# Autodesk Inventor assembly: 2016_IEEE_SouteastCon_Court final
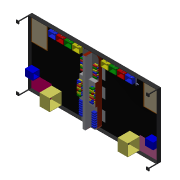
[picture p0: Inventor's stored thumbnail of the model, 180x180]
Saved by Autodesk Inventor 2015 (Build 190159000, 159)
## iProperties
Created: 2015-03-03
Part Number: 2016_IEEE_SouteastCon_Court final
Document SubType Name: Assembly
Designer: Vukica
Author: Vukica
## Documents named in this file (17)
- C:\Users\Vukica\Dropbox\IEEE\hardware rules\2016Hardware_Court_v6\2016_IEEE_SouteastCon_Court final.iam
- C:\Users\Vukica\Dropbox\IEEE\hardware rules\2016Hardware_Court_v6\Base.ipt
- C:\Users\Vukica\Dropbox\IEEE\hardware rules\2016Hardware_Court_v6\Ship area.ipt
- C:\Users\Vukica\Dropbox\IEEE\hardware rules\2016Hardware_Court_v6\Starting position pink.ipt
- C:\Users\Vukica\Dropbox\IEEE\hardware rules\2016Hardware_Court_v6\Starting position purple.ipt
- C:\Users\Vukica\Dropbox\IEEE\hardware rules\2016Hardware_Court_v6\Beacon.ipt
- C:\Users\Vukica\Dropbox\IEEE\hardware rules\2016Hardware_Court_v6\Side 84 in by 6 in by half inch.ipt
- C:\Users\Vukica\Dropbox\IEEE\hardware rules\2016Hardware_Court_v6\Side 120 in by 6 in by half inch.ipt
- C:\Users\Vukica\Dropbox\IEEE\hardware rules\2016Hardware_Court_v6\Hill.ipt
- C:\Users\Vukica\Dropbox\IEEE\hardware rules\2016Hardware_Court_v6\Blue truck.ipt
- C:\Users\Vukica\Dropbox\IEEE\hardware rules\2016Hardware_Court_v6\Tunnel.ipt
- C:\Users\Vukica\Dropbox\IEEE\hardware rules\2016Hardware_Court_v6\Shipping goods QR subassembly.iam
- C:\Users\Vukica\Dropbox\IEEE\hardware rules\2016Hardware_Court_v6\Shipping goods generic subassembly.iam
- C:\Users\Vukica\Dropbox\IEEE\hardware rules\2016Hardware_Court_v6\Shipping goods colors subassembly.iam
- C:\Users\Vukica\Dropbox\IEEE\hardware rules\2016Hardware_Court_v6\Rail truck area subassembly v2.iam
- C:\Users\Vukica\Dropbox\IEEE\hardware rules\2016Hardware_Court_v6\LED Bacon.iam
- C:\Users\Vukica\Dropbox\IEEE\hardware rules\2016Hardware_Court_v6\Stripes on the floor.ipt
## Components (31 placed, 16 different names)
1. Base:1 — Mate:1, Mate:2, Mate:3, Flush:5, Flush:6, Mate:4, Flush:7, Flush:8, Flush:11, Mate:9, Flush:12, Flush:13, Flush:15, Mate:10, Mate:11, Flush:16, Flush:18, Mate:12, Mate:17, Mate:22, Mate:30, Mate:62, Mate:125, Mate:126, Mate:127, Mate:136, Mate:137, Flush:55, Flush:56
2. Ship area:1 — Mate:1, Mate:118, Mate:119
3. Ship area:2 — Mate:2, Mate:120, Mate:121
4. Starting position pink:1 — Mate:4, Flush:7, Flush:8, Mate:128, Mate:135
5. Starting position purple:1 — Mate:3, Flush:5, Flush:6, Mate:130, Mate:133
6. Beacon:1 — Mate:14, Flush:22, Flush:23
7. Beacon:2 — Mate:13, Flush:20, Flush:21
8. Beacon:3 — Mate:15, Flush:24, Flush:25
9. Beacon:4 — Mate:16, Flush:26, Flush:27
10. Side 84 in by 6 in by half inch:1 — Mate:11, Flush:16, Flush:17, Mate:15, Flush:25, Mate:16, Flush:26, Flush:27, Flush:51, Mate:120, Mate:134
11. Side 84 in by 6 in by half inch:2 — Flush:18, Mate:12, Flush:19, Mate:13, Flush:21, Mate:14, Flush:23, Mate:119, Mate:132
12. Side 120 in by 6 in by half inch:1 — Flush:13, Flush:15, Mate:10, Flush:17, Flush:22, Flush:24, Mate:118, Mate:121, Mate:138, Mate:140
13. Side 120 in by 6 in by half inch:2 — Flush:11, Mate:9, Flush:12, Flush:19, Flush:20, Mate:84, Mate:129, Mate:131
14. Barge:1 — Mate:17, Mate:84, Mate:94, Flush:44, Mate:95, Mate:96, Mate:97, Flush:47, Mate:98, Flush:48, Mate:99, Mate:100, Flush:49, Mate:101, Mate:102, Flush:50, Mate:103, Flush:51, Flush:52, Mate:139, Mate:141, Flush:53, Flush:54, Mate:142, Mate:143, Mate:144, Mate:145, Mate:146, Mate:147, Mate:148, Mate:149, Mate:150, Mate:151, Mate:152, Mate:153
15. Blue truck:1 — Mate:22, Mate:132, Mate:133
16. Blue truck:2 — Mate:30, Mate:134, Mate:135
17. Tunnel:1 — Mate:62, Mate:126, Mate:127, Mate:128, Mate:129
18. Shipping goods QR subassembly:1 [sub-assembly] — Mate:94, Flush:44, Flush:52
19. Shipping goods QR subassembly:2 [sub-assembly] — Mate:95, Flush:53, Flush:54
20. Shipping goods generic subassembly:1 [sub-assembly] — Mate:96, Mate:97, Flush:47
21. Shipping goods generic subassembly:2 [sub-assembly] — Mate:98, Flush:48, Mate:99
22. Shipping goods colors subassembly:1 [sub-assembly] — Mate:102, Flush:50, Mate:103
23. Shipping goods colors subassembly:2 [sub-assembly] — Mate:100, Flush:49, Mate:101
24. Tunnel:2 — Mate:125, Mate:130, Mate:131
25. Rail truck area subassembly v2:1 [sub-assembly] — Mate:136, Mate:140, Mate:141
26. Rail truck area subassembly v2:2 [sub-assembly] — Mate:137, Mate:138, Mate:139
27. LED Bacon:1 [sub-assembly] — Mate:142, Mate:143, Mate:144
28. LED Bacon:2 [sub-assembly] — Mate:145, Mate:146, Mate:147
29. LED Bacon:3 [sub-assembly] — Mate:148, Mate:149, Mate:150
30. LED Bacon:4 [sub-assembly] — Mate:151, Mate:152, Mate:153
31. Stripes on the floor:1 — Flush:55, Flush:56
## Relationships (91: Mate 60, Flush 31)
- Mate:1: Base:1 ↔ Ship area:1
- Mate:2: Base:1 ↔ Ship area:2
- Mate:3: Base:1 ↔ Starting position purple:1
- Flush:5: Base:1 ↔ Starting position purple:1
- Flush:6: Base:1 ↔ Starting position purple:1
- Mate:4: Base:1 ↔ Starting position pink:1
- Flush:7: Base:1 ↔ Starting position pink:1
- Flush:8: Base:1 ↔ Starting position pink:1
- Flush:11: Base:1 ↔ Side 120 in by 6 in by half inch:2
- Mate:9: Base:1 ↔ Side 120 in by 6 in by half inch:2
- Flush:12: Base:1 ↔ Side 120 in by 6 in by half inch:2
- Flush:13: Base:1 ↔ Side 120 in by 6 in by half inch:1
- Flush:15: Base:1 ↔ Side 120 in by 6 in by half inch:1
- Mate:10: Base:1 ↔ Side 120 in by 6 in by half inch:1
- Mate:11: Base:1 ↔ Side 84 in by 6 in by half inch:1
- Flush:16: Base:1 ↔ Side 84 in by 6 in by half inch:1
- Flush:17: Side 84 in by 6 in by half inch:1 ↔ Side 120 in by 6 in by half inch:1
- Flush:18: Base:1 ↔ Side 84 in by 6 in by half inch:2
- Mate:12: Base:1 ↔ Side 84 in by 6 in by half inch:2
- Flush:19: Side 84 in by 6 in by half inch:2 ↔ Side 120 in by 6 in by half inch:2
- Mate:13: Beacon:2 ↔ Side 84 in by 6 in by half inch:2
- Flush:20: Beacon:2 ↔ Side 120 in by 6 in by half inch:2
- Flush:21: Beacon:2 ↔ Side 84 in by 6 in by half inch:2
- Mate:14: Beacon:1 ↔ Side 84 in by 6 in by half inch:2
- Flush:22: Beacon:1 ↔ Side 120 in by 6 in by half inch:1
- Flush:23: Beacon:1 ↔ Side 84 in by 6 in by half inch:2
- Mate:15: Beacon:3 ↔ Side 84 in by 6 in by half inch:1
- Flush:24: Beacon:3 ↔ Side 120 in by 6 in by half inch:1
- Flush:25: Beacon:3 ↔ Side 84 in by 6 in by half inch:1
- Mate:16: Beacon:4 ↔ Side 84 in by 6 in by half inch:1
- Flush:26: Beacon:4 ↔ Side 84 in by 6 in by half inch:1
- Flush:27: Beacon:4 ↔ Side 84 in by 6 in by half inch:1
- Mate:17: Base:1 ↔ Barge:1
- Mate:22: Base:1 ↔ Blue truck:1
- Mate:30: Base:1 ↔ Blue truck:2
- Mate:62: Base:1 ↔ Tunnel:1
- Mate:84: Side 120 in by 6 in by half inch:2 ↔ Barge:1
- Mate:94: Barge:1 ↔ Shipping goods QR subassembly:1
- Flush:44: Barge:1 ↔ Shipping goods QR subassembly:1
- Mate:95: Barge:1 ↔ Shipping goods QR subassembly:2
- Mate:96: Barge:1 ↔ Shipping goods generic subassembly:1
- Mate:97 (25.4 mm): Barge:1 ↔ Shipping goods generic subassembly:1
- Flush:47: Barge:1 ↔ Shipping goods generic subassembly:1
- Mate:98: Barge:1 ↔ Shipping goods generic subassembly:2
- Flush:48: Barge:1 ↔ Shipping goods generic subassembly:2
- Mate:99 (25.4 mm): Barge:1 ↔ Shipping goods generic subassembly:2
- Mate:100: Barge:1 ↔ Shipping goods colors subassembly:2
- Flush:49: Barge:1 ↔ Shipping goods colors subassembly:2
- Mate:101 (101.6 mm): Barge:1 ↔ Shipping goods colors subassembly:2
- Mate:102: Barge:1 ↔ Shipping goods colors subassembly:1
- Flush:50: Barge:1 ↔ Shipping goods colors subassembly:1
- Mate:103 (101.6 mm): Barge:1 ↔ Shipping goods colors subassembly:1
- Flush:51 (2209.8 mm): Side 84 in by 6 in by half inch:1 ↔ Barge:1
- Mate:118: Ship area:1 ↔ Side 120 in by 6 in by half inch:1
- Mate:119: Ship area:1 ↔ Side 84 in by 6 in by half inch:2
- Mate:120: Ship area:2 ↔ Side 84 in by 6 in by half inch:1
- Mate:121: Ship area:2 ↔ Side 120 in by 6 in by half inch:1
- Mate:125: Base:1 ↔ Tunnel:2
- Mate:126: Base:1 ↔ Tunnel:1
- Mate:127: Base:1 ↔ Tunnel:1
- Mate:128: Starting position pink:1 ↔ Tunnel:1
- Mate:129: Side 120 in by 6 in by half inch:2 ↔ Tunnel:1
- Mate:130: Starting position purple:1 ↔ Tunnel:2
- Mate:131: Side 120 in by 6 in by half inch:2 ↔ Tunnel:2
- Mate:132: Side 84 in by 6 in by half inch:2 ↔ Blue truck:1
- Mate:133: Starting position purple:1 ↔ Blue truck:1
- Mate:134: Side 84 in by 6 in by half inch:1 ↔ Blue truck:2
- Mate:135: Starting position pink:1 ↔ Blue truck:2
- Flush:52 (152.4 mm): Barge:1 ↔ Shipping goods QR subassembly:1
- Mate:136: Base:1 ↔ Rail truck area subassembly v2:1
- Mate:137: Base:1 ↔ Rail truck area subassembly v2:2
- Mate:138: Side 120 in by 6 in by half inch:1 ↔ Rail truck area subassembly v2:2
- Mate:139: Barge:1 ↔ Rail truck area subassembly v2:2
- Mate:140: Side 120 in by 6 in by half inch:1 ↔ Rail truck area subassembly v2:1
- Mate:141: Barge:1 ↔ Rail truck area subassembly v2:1
- Flush:53 (152.4 mm): Barge:1 ↔ Shipping goods QR subassembly:2
- Flush:54: Barge:1 ↔ Shipping goods QR subassembly:2
- Mate:142 (-12.7 mm): Barge:1 ↔ LED Bacon:1
- Mate:143: Barge:1 ↔ LED Bacon:1
- Mate:144: Barge:1 ↔ LED Bacon:1
- Mate:145 (-12.7 mm): Barge:1 ↔ LED Bacon:2
- Mate:146: Barge:1 ↔ LED Bacon:2
- Mate:147: Barge:1 ↔ LED Bacon:2
- Mate:148 (-12.7 mm): Barge:1 ↔ LED Bacon:3
- Mate:149: Barge:1 ↔ LED Bacon:3
- Mate:150: Barge:1 ↔ LED Bacon:3
- Mate:151 (-12.7 mm): Barge:1 ↔ LED Bacon:4
- Mate:152: Barge:1 ↔ LED Bacon:4
- Mate:153: Barge:1 ↔ LED Bacon:4
- Flush:55: Base:1 ↔ Stripes on the floor:1
- Flush:56: Base:1 ↔ Stripes on the floor:1
